# Autodesk Inventor assembly: PodFloorSubAssembly
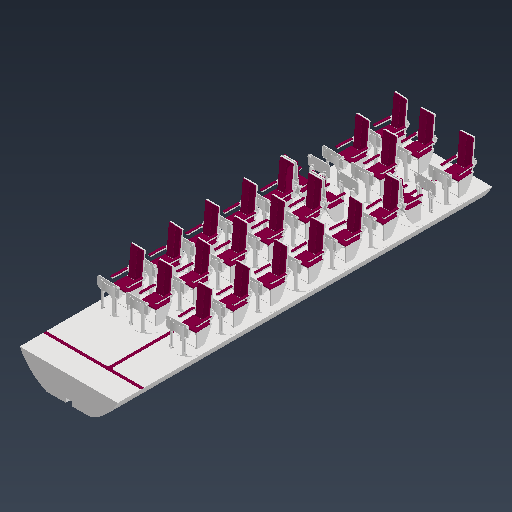
[picture p0: Inventor's stored thumbnail of the model, 512x512]
Saved by Autodesk Inventor 2021 (Build 250183000, 183)
## iProperties
Created: 2021-01-31
Part Number: PodFloorSubAssembly
Document SubType Name: Assembly
Designer: argon
Author: argon
## Documents named in this file (4)
- C:\Users\argon\OneDrive\Documents\GrabCAD\EngOne Maroons\Pod Subassembly\PodFloorSubAssembly.iam
- C:\Users\argon\OneDrive\Documents\GrabCAD\EngOne Maroons\Pod Subassembly\Floor.ipt
- C:\Users\argon\OneDrive\Documents\GrabCAD\EngOne Maroons\Seat Module Subassembly\SeatModuleSubassembly.iam
- C:\Users\argon\OneDrive\Documents\GrabCAD\EngOne Maroons\Pod Subassembly\FloorStripe.ipt
## Components (26 placed, 3 different names)
1. Floor:1 — Mate:1, Mate:2, Mate:4, Mate:5, Mate:6, Mate:7, Mate:8, Mate:9, Mate:10, Mate:11, Mate:12, Mate:13, Mate:14, Mate:15, Mate:16, Mate:17, Mate:18, Mate:19, Mate:20, Mate:21, Mate:22, Mate:23, Mate:24, Mate:25, Mate:26, Mate:27, Mate:28, Mate:29, Mate:30, Mate:31, Mate:32, Mate:33, Mate:34, Mate:35, Mate:36, Mate:37, Mate:38, Mate:39, Mate:40, Mate:41, Mate:42, Mate:43, Mate:44, Mate:45, Mate:46, Mate:47, Mate:48, Mate:49, Mate:50, Mate:51, Mate:52
2. SeatModuleSubassembly:1 [sub-assembly] — Mate:2, Mate:5
3. SeatModuleSubassembly:3 [sub-assembly] — Mate:12, Mate:13
4. SeatModuleSubassembly:4 [sub-assembly] — Mate:1, Mate:4
5. SeatModuleSubassembly:5 [sub-assembly] — Mate:9, Mate:10
6. SeatModuleSubassembly:6 [sub-assembly] — Mate:14, Mate:15
7. SeatModuleSubassembly:7 [sub-assembly] — Mate:16, Mate:17
8. SeatModuleSubassembly:8 [sub-assembly] — Mate:8, Mate:11
9. SeatModuleSubassembly:9 [sub-assembly] — Mate:6, Mate:7
10. SeatModuleSubassembly:10 [sub-assembly] — Mate:18, Mate:19
11. SeatModuleSubassembly:11 [sub-assembly] — Mate:20, Mate:25
12. SeatModuleSubassembly:12 [sub-assembly] — Mate:21, Mate:23
13. SeatModuleSubassembly:13 [sub-assembly] — Mate:22, Mate:24
14. SeatModuleSubassembly:14 [sub-assembly] — Mate:28, Mate:30
15. SeatModuleSubassembly:15 [sub-assembly] — Mate:26, Mate:32
16. SeatModuleSubassembly:16 [sub-assembly] — Mate:29, Mate:31
17. SeatModuleSubassembly:17 [sub-assembly] — Mate:27, Mate:33
18. SeatModuleSubassembly:18 [sub-assembly] — Mate:34, Mate:35
19. SeatModuleSubassembly:19 [sub-assembly] — Mate:38, Mate:39
20. SeatModuleSubassembly:20 [sub-assembly] — Mate:36, Mate:37
21. SeatModuleSubassembly:21 [sub-assembly] — Mate:40, Mate:41
22. SeatModuleSubassembly:22 [sub-assembly] — Mate:42, Mate:43
23. SeatModuleSubassembly:23 [sub-assembly] — Mate:44, Mate:45
24. SeatModuleSubassembly:24 [sub-assembly] — Mate:46, Mate:49
25. SeatModuleSubassembly:25 [sub-assembly] — Mate:47, Mate:48
26. FloorStripe:1 — Mate:50, Mate:51, Mate:52
## Relationships (51: Mate 51)
- Mate:1: Floor:1 ↔ SeatModuleSubassembly:4
- Mate:2: Floor:1 ↔ SeatModuleSubassembly:1
- Mate:4: Floor:1 ↔ SeatModuleSubassembly:4
- Mate:5: Floor:1 ↔ SeatModuleSubassembly:1
- Mate:6: Floor:1 ↔ SeatModuleSubassembly:9
- Mate:7: Floor:1 ↔ SeatModuleSubassembly:9
- Mate:8: Floor:1 ↔ SeatModuleSubassembly:8
- Mate:9: Floor:1 ↔ SeatModuleSubassembly:5
- Mate:10: Floor:1 ↔ SeatModuleSubassembly:5
- Mate:11: Floor:1 ↔ SeatModuleSubassembly:8
- Mate:12: Floor:1 ↔ SeatModuleSubassembly:3
- Mate:13: Floor:1 ↔ SeatModuleSubassembly:3
- Mate:14: Floor:1 ↔ SeatModuleSubassembly:6
- Mate:15: Floor:1 ↔ SeatModuleSubassembly:6
- Mate:16: Floor:1 ↔ SeatModuleSubassembly:7
- Mate:17: Floor:1 ↔ SeatModuleSubassembly:7
- Mate:18: Floor:1 ↔ SeatModuleSubassembly:10
- Mate:19: Floor:1 ↔ SeatModuleSubassembly:10
- Mate:20: Floor:1 ↔ SeatModuleSubassembly:11
- Mate:21: Floor:1 ↔ SeatModuleSubassembly:12
- Mate:22: Floor:1 ↔ SeatModuleSubassembly:13
- Mate:23: Floor:1 ↔ SeatModuleSubassembly:12
- Mate:24: Floor:1 ↔ SeatModuleSubassembly:13
- Mate:25: Floor:1 ↔ SeatModuleSubassembly:11
- Mate:26: Floor:1 ↔ SeatModuleSubassembly:15
- Mate:27: Floor:1 ↔ SeatModuleSubassembly:17
- Mate:28: Floor:1 ↔ SeatModuleSubassembly:14
- Mate:29: Floor:1 ↔ SeatModuleSubassembly:16
- Mate:30: Floor:1 ↔ SeatModuleSubassembly:14
- Mate:31: Floor:1 ↔ SeatModuleSubassembly:16
- Mate:32: Floor:1 ↔ SeatModuleSubassembly:15
- Mate:33: Floor:1 ↔ SeatModuleSubassembly:17
- Mate:34: Floor:1 ↔ SeatModuleSubassembly:18
- Mate:35: Floor:1 ↔ SeatModuleSubassembly:18
- Mate:36: Floor:1 ↔ SeatModuleSubassembly:20
- Mate:37: Floor:1 ↔ SeatModuleSubassembly:20
- Mate:38: Floor:1 ↔ SeatModuleSubassembly:19
- Mate:39: Floor:1 ↔ SeatModuleSubassembly:19
- Mate:40: Floor:1 ↔ SeatModuleSubassembly:21
- Mate:41: Floor:1 ↔ SeatModuleSubassembly:21
- Mate:42: Floor:1 ↔ SeatModuleSubassembly:22
- Mate:43: Floor:1 ↔ SeatModuleSubassembly:22
- Mate:44: Floor:1 ↔ SeatModuleSubassembly:23
- Mate:45: Floor:1 ↔ SeatModuleSubassembly:23
- Mate:46: Floor:1 ↔ SeatModuleSubassembly:24
- Mate:47: Floor:1 ↔ SeatModuleSubassembly:25
- Mate:48: Floor:1 ↔ SeatModuleSubassembly:25
- Mate:49: Floor:1 ↔ SeatModuleSubassembly:24
- Mate:50: Floor:1 ↔ FloorStripe:1
- Mate:51: Floor:1 ↔ FloorStripe:1
- Mate:52: Floor:1 ↔ FloorStripe:1
